# Autodesk Inventor assembly: Heat Exchanger
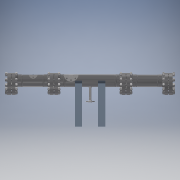
[picture p0: Inventor's stored thumbnail of the model, 180x180]
Saved by Autodesk Inventor 2016 (Build 200138000, 138)
## iProperties
Created: 2018-11-05
Part Number: Heat Exchanger
Document SubType Name: Weldment
Designer: Wijaya
Weld Material: Steel, Carbon
Mass: 1.24439e+06 g
Surface Area: 233524 cm^2
Volume: 160879 cm^3
Density: 7.73496 g/cm^3
_SolveAssemblyDoc: Frame Generator Solve Assembly
_Version: 15.0.0
Author: Wijaya
## Documents named in this file (30)
- C:\Users\Wijaya\Documents\Inventor\Medcom\Heat Exchanger.iam
- C:\Users\Wijaya\Documents\Inventor\Medcom\Shell Pipe.ipt
- C:\Users\Wijaya\Documents\Inventor\Medcom\Weldneck Flange 14 in.ipt
- C:\Users\Wijaya\Documents\Inventor\Medcom\Front Head Pipe.ipt
- C:\Users\Wijaya\Documents\Inventor\Content Center Files\R2016\en-US\ASTM F436(1)\ASTM F436 - 1 1_8(1).ipt
- C:\Users\Wijaya\Documents\Inventor\Medcom\Blind Flange 14 in.ipt
- C:\Users\Wijaya\Documents\Inventor\Medcom\Gasket.ipt
- C:\Users\Wijaya\Documents\Inventor\Medcom\Rear Head Pipe.ipt
- C:\Users\Wijaya\Documents\Inventor\Medcom\Lifting Lug.ipt
- C:\Users\Wijaya\Documents\Inventor\Medcom\Fix Saddle.ipt
- C:\Users\Wijaya\Documents\Inventor\Medcom\Slidding Saddle.ipt
- C:\Users\Wijaya\Documents\Inventor\Medcom\Tube.ipt
- C:\Users\Wijaya\Documents\Inventor\Medcom\Tube Sheet.ipt
- C:\Users\Wijaya\Documents\Inventor\Medcom\Heat Exchanger\Frame\Frame0002.iam
- C:\Users\Wijaya\Documents\Inventor\Medcom\Heat Exchanger\Frame\Frame00021.iam
- C:\Users\Wijaya\Documents\Inventor\Medcom\Tie Rod.ipt
- C:\Users\Wijaya\Documents\Inventor\Medcom\Flange 3 in.ipt
- C:\Users\Wijaya\Documents\Inventor\Medcom\Flange 1 in.ipt
- C:\Users\Wijaya\Documents\Inventor\Medcom\Plate Partition.ipt
- C:\Users\Wijaya\Documents\Inventor\Medcom\Nozzle Pipe 3 in.ipt
- C:\Users\Wijaya\Documents\Inventor\Medcom\Nozzle Pipe 1 in.ipt
- C:\Users\Wijaya\Documents\Inventor\Medcom\Nozzle Pipe 1 in drain.ipt
- C:\Users\Wijaya\Documents\Inventor\Medcom\DIN 976-1 - M30 x 180 - A.ipt
- C:\Users\Wijaya\Documents\Inventor\Medcom\DIN 6915 - M30.ipt
- C:\Users\Wijaya\Documents\Inventor\Medcom\Heat Exchanger\AIP\FEA\cpcsafi80.fins
- C:\Users\Wijaya\Documents\Inventor\Medcom\Heat Exchanger\AIP\FEA\cpcsafi80.fsat
- C:\Users\Wijaya\Documents\Inventor\Medcom\Heat Exchanger\AIP\FEA\cpcsafi80.ftes
- C:\Users\Wijaya\Documents\Inventor\Medcom\Heat Exchanger\AIP\FEA\cpcsafi80.fwiz
- C:\Users\Wijaya\Documents\Inventor\Medcom\Heat Exchanger\AIP\FEA\cpcsafj28.fmsh
- C:\Users\Wijaya\Documents\Inventor\Medcom\Heat Exchanger\AIP\FEA\cpcsafj29.fres
## Components (439 placed, 23 different names)
1. Shell Pipe:1 — Mate:3, Mate:4, Mate:12, Mate:14, Mate:15, Mate:18, Mate:19, Mate:42, Mate:61, Mate:77, Mate:78, Mate:79, Mate:80, Mate:101, Flush:1, Mate:103, Flush:2, Mate:106, Mate:107, Mate:108, Mate:109, Mate:117, Mate:118, Mate:119, Mate:120, Mate:141, Mate:142, Mate:146, Mate:147, Mate:161, Mate:162
2. Weldneck Flange 14 in:1 — Mate:118, Mate:119, Mate:120, Mate:121, Mate:122, Flush:6, Mate:123, Symmetry:5, Rotational:8
3. Weldneck Flange 14 in:2 — Mate:3, Mate:4, Mate:14, Rotational:1, Symmetry:3, Mate:116, Mate:182, Rotational:9
4. Nozzle Pipe 3 in:1 — Mate:141, Mate:142, Mate:143, Mate:144, Mate:145
5. Nozzle Pipe 3 in:2 — Mate:146, Mate:147, Mate:148, Mate:149, Mate:150
6. Nozzle Pipe 1 in drain:1 — Mate:161, Mate:162, Mate:163, Mate:164, Mate:165
7. Flange 3 in:1 — Mate:143, Mate:144, Mate:145
8. Flange 3 in:2 — Mate:148, Mate:149, Mate:150
9. Flange 1 in:3 — Mate:163, Mate:164, Mate:165
10. Plate Partition:1 — Mate:139, Mate:140, Mate:198
11. Gasket:1 — Mate:42, Mate:43, Mate:123
12. Gasket:3 — Rotational:1, Rotational:2
13. Front Head Pipe:1 — Mate:10, Mate:11, Mate:12, Mate:16, Mate:17, Mate:19, Mate:139, Mate:140, Mate:151, Mate:152, Mate:156, Mate:157
14. Weldneck Flange 14 in:3 — Mate:15, Mate:16, Mate:17, Mate:33, Mate:44, Mate:45, Mate:60, Symmetry:2, Mate:170, Mate:173
15. Weldneck Flange 14 in:4 — Mate:10, Mate:11, Mate:18, Mate:43, Mate:174, Symmetry:5, Rotational:7, Mate:180, Mate:181
16. Blind Flange 14 in:1 — Mate:60, Mate:61, Mate:62, Symmetry:2, Mate:65, Mate:166, Mate:198
17. Nozzle Pipe 1 in:1 — Mate:151, Mate:152, Mate:153, Mate:154, Mate:155
18. Nozzle Pipe 1 in:2 — Mate:156, Mate:157, Mate:158, Mate:159, Mate:160
19. Flange 1 in:1 — Mate:153, Mate:154, Mate:155
20. Flange 1 in:2 — Mate:158, Mate:159, Mate:160
21. Gasket:2 — Mate:44, Mate:45, Mate:62
22. Rear Head Pipe:1 — Rotational:3, Rotational:4, Mate:80
23. Weldneck Flange 14 in:5 — Rotational:2, Rotational:3, Mate:77, Symmetry:3, Rotational:10, Mate:186, Mate:189
24. Weldneck Flange 14 in:6 — Rotational:4, Rotational:5, Mate:78, Symmetry:4, Mate:190, Rotational:11, Mate:196, Mate:197
25. Blind Flange 14 in:2 — Rotational:6, Mate:79, Symmetry:4, Rotational:12
26. Gasket:4 — Rotational:5, Rotational:6
27. Lifting Lug:1 — Mate:101, Flush:1, Mate:102
28. Lifting Lug:2 — Mate:103, Flush:2, Mate:104
29. Fix Saddle:1 — Mate:106, Mate:108, Mate:110
30. Slidding Saddle:1 — Mate:107, Mate:109, Mate:111
31. Tube Sheet:1 — Mate:116, Mate:117, Flush:5
32. Tube Sheet:2 — Mate:121, Mate:122, Flush:6, Mate:124, Flush:7
33. Tube:1 — Flush:5
34. Frame0002:1 [sub-assembly]
35. Frame00021:1 [sub-assembly]
36. Tie Rod:1 — Mate:124, Flush:7
37. Tie Rod:2
38. Tie Rod:3
39. Tie Rod:4
40. DIN 976-1 A M30 x 180:1 — Mate:166, Mate:167, Mate:168, Mate:171
41. DIN 6915 M30:1 — Mate:171, Mate:172, Mate:173
42. DIN 6915 M30:2 — Mate:168, Mate:169, Mate:170
43. Circular Washer (Inch) 1 1/8:41 — Mate:33, Mate:169
44. Circular Washer (Inch) 1 1/8:43 — Mate:65, Mate:172
45. DIN 976-1 A M30 x 180:2
46. DIN 6915 M30:3
47. DIN 6915 M30:4
48. Circular Washer (Inch) 1 1/8:44
49. Circular Washer (Inch) 1 1/8:45
50. DIN 976-1 A M30 x 180:3
51. DIN 6915 M30:5
52. DIN 6915 M30:6
53. Circular Washer (Inch) 1 1/8:46
54. Circular Washer (Inch) 1 1/8:47
55. DIN 976-1 A M30 x 180:4
56. DIN 6915 M30:7
57. DIN 6915 M30:8
58. Circular Washer (Inch) 1 1/8:48
59. Circular Washer (Inch) 1 1/8:49
60. DIN 976-1 A M30 x 180:5
61. DIN 6915 M30:9
62. DIN 6915 M30:10
63. Circular Washer (Inch) 1 1/8:50
64. Circular Washer (Inch) 1 1/8:51
65. DIN 976-1 A M30 x 180:6
66. DIN 6915 M30:11
67. DIN 6915 M30:12
68. Circular Washer (Inch) 1 1/8:52
69. Circular Washer (Inch) 1 1/8:53
70. DIN 976-1 A M30 x 180:7
71. DIN 6915 M30:13
72. DIN 6915 M30:14
73. Circular Washer (Inch) 1 1/8:54
74. Circular Washer (Inch) 1 1/8:55
75. DIN 976-1 A M30 x 180:8
76. DIN 6915 M30:15
77. DIN 6915 M30:16
78. Circular Washer (Inch) 1 1/8:56
79. Circular Washer (Inch) 1 1/8:57
80. DIN 976-1 A M30 x 180:9
81. DIN 6915 M30:17
82. DIN 6915 M30:18
83. Circular Washer (Inch) 1 1/8:58
84. Circular Washer (Inch) 1 1/8:59
85. DIN 976-1 A M30 x 180:10
86. DIN 6915 M30:19
87. DIN 6915 M30:20
88. Circular Washer (Inch) 1 1/8:60
89. Circular Washer (Inch) 1 1/8:61
90. DIN 976-1 A M30 x 180:11
91. DIN 6915 M30:21
92. DIN 6915 M30:22
93. Circular Washer (Inch) 1 1/8:62
94. Circular Washer (Inch) 1 1/8:63
95. DIN 976-1 A M30 x 180:12
96. DIN 6915 M30:23
97. DIN 6915 M30:24
98. Circular Washer (Inch) 1 1/8:64
99. Circular Washer (Inch) 1 1/8:65
100. DIN 976-1 A M30 x 180:13
101. DIN 6915 M30:25
102. DIN 6915 M30:26
103. Circular Washer (Inch) 1 1/8:66
104. Circular Washer (Inch) 1 1/8:67
105. DIN 976-1 A M30 x 180:14
106. DIN 6915 M30:27
107. DIN 6915 M30:28
108. Circular Washer (Inch) 1 1/8:68
109. Circular Washer (Inch) 1 1/8:69
110. DIN 976-1 A M30 x 180:15
111. DIN 6915 M30:29
112. DIN 6915 M30:30
113. Circular Washer (Inch) 1 1/8:70
114. Circular Washer (Inch) 1 1/8:71
115. DIN 976-1 A M30 x 180:16
116. DIN 6915 M30:31
117. DIN 6915 M30:32
118. Circular Washer (Inch) 1 1/8:72
119. Circular Washer (Inch) 1 1/8:73
120. DIN 976-1 A M30 x 180:17
121. DIN 6915 M30:33
122. DIN 6915 M30:34
123. Circular Washer (Inch) 1 1/8:74
124. Circular Washer (Inch) 1 1/8:75
125. DIN 976-1 A M30 x 180:18
126. DIN 6915 M30:35
127. DIN 6915 M30:36
128. Circular Washer (Inch) 1 1/8:76
129. Circular Washer (Inch) 1 1/8:77
130. DIN 976-1 A M30 x 180:19
131. DIN 6915 M30:37
132. DIN 6915 M30:38
133. Circular Washer (Inch) 1 1/8:78
134. Circular Washer (Inch) 1 1/8:79
135. DIN 976-1 A M30 x 180:20
136. DIN 6915 M30:39
137. DIN 6915 M30:40
138. Circular Washer (Inch) 1 1/8:80
139. Circular Washer (Inch) 1 1/8:81
140. DIN 976-1 A M30 x 180:21 — Mate:174, Mate:175, Mate:176, Mate:177
141. DIN 6915 M30:41 — Mate:176, Mate:179, Mate:180
142. DIN 6915 M30:42 — Mate:177, Mate:178, Mate:181
143. Circular Washer (Inch) 1 1/8:82 — Rotational:7, Mate:179
144. Circular Washer (Inch) 1 1/8:83 — Rotational:8, Mate:178
145. DIN 976-1 A M30 x 180:24
146. DIN 6915 M30:47
147. DIN 6915 M30:48
148. Circular Washer (Inch) 1 1/8:88
149. Circular Washer (Inch) 1 1/8:89
150. DIN 976-1 A M30 x 180:25
151. DIN 6915 M30:49
152. DIN 6915 M30:50
153. Circular Washer (Inch) 1 1/8:90
154. Circular Washer (Inch) 1 1/8:91
155. DIN 976-1 A M30 x 180:26
156. DIN 6915 M30:51
157. DIN 6915 M30:52
158. Circular Washer (Inch) 1 1/8:92
159. Circular Washer (Inch) 1 1/8:93
160. DIN 976-1 A M30 x 180:27
161. DIN 6915 M30:53
162. DIN 6915 M30:54
163. Circular Washer (Inch) 1 1/8:94
164. Circular Washer (Inch) 1 1/8:95
165. DIN 976-1 A M30 x 180:28
166. DIN 6915 M30:55
167. DIN 6915 M30:56
168. Circular Washer (Inch) 1 1/8:96
169. Circular Washer (Inch) 1 1/8:97
170. DIN 976-1 A M30 x 180:29
171. DIN 6915 M30:57
172. DIN 6915 M30:58
173. Circular Washer (Inch) 1 1/8:98
174. Circular Washer (Inch) 1 1/8:99
175. DIN 976-1 A M30 x 180:30
176. DIN 6915 M30:59
177. DIN 6915 M30:60
178. Circular Washer (Inch) 1 1/8:100
179. Circular Washer (Inch) 1 1/8:101
180. DIN 976-1 A M30 x 180:31
181. DIN 6915 M30:61
182. DIN 6915 M30:62
183. Circular Washer (Inch) 1 1/8:102
184. Circular Washer (Inch) 1 1/8:103
185. DIN 976-1 A M30 x 180:32
186. DIN 6915 M30:63
187. DIN 6915 M30:64
188. Circular Washer (Inch) 1 1/8:104
189. Circular Washer (Inch) 1 1/8:105
190. DIN 976-1 A M30 x 180:33
191. DIN 6915 M30:65
192. DIN 6915 M30:66
193. Circular Washer (Inch) 1 1/8:106
194. Circular Washer (Inch) 1 1/8:107
195. DIN 976-1 A M30 x 180:34
196. DIN 6915 M30:67
197. DIN 6915 M30:68
198. Circular Washer (Inch) 1 1/8:108
199. Circular Washer (Inch) 1 1/8:109
200. DIN 976-1 A M30 x 180:35
201. DIN 6915 M30:69
202. DIN 6915 M30:70
203. Circular Washer (Inch) 1 1/8:110
204. Circular Washer (Inch) 1 1/8:111
205. DIN 976-1 A M30 x 180:36
206. DIN 6915 M30:71
207. DIN 6915 M30:72
208. Circular Washer (Inch) 1 1/8:112
209. Circular Washer (Inch) 1 1/8:113
210. DIN 976-1 A M30 x 180:37
211. DIN 6915 M30:73
212. DIN 6915 M30:74
213. Circular Washer (Inch) 1 1/8:114
214. Circular Washer (Inch) 1 1/8:115
215. DIN 976-1 A M30 x 180:38
216. DIN 6915 M30:75
217. DIN 6915 M30:76
218. Circular Washer (Inch) 1 1/8:116
219. Circular Washer (Inch) 1 1/8:117
220. DIN 976-1 A M30 x 180:39
221. DIN 6915 M30:77
222. DIN 6915 M30:78
223. Circular Washer (Inch) 1 1/8:118
224. Circular Washer (Inch) 1 1/8:119
225. DIN 976-1 A M30 x 180:40
226. DIN 6915 M30:79
227. DIN 6915 M30:80
228. Circular Washer (Inch) 1 1/8:120
229. Circular Washer (Inch) 1 1/8:121
230. DIN 976-1 A M30 x 180:41
231. DIN 6915 M30:81
232. DIN 6915 M30:82
233. Circular Washer (Inch) 1 1/8:122
234. Circular Washer (Inch) 1 1/8:123
235. DIN 976-1 A M30 x 180:42
236. DIN 6915 M30:83
237. DIN 6915 M30:84
238. Circular Washer (Inch) 1 1/8:124
239. Circular Washer (Inch) 1 1/8:125
240. Circular Washer (Inch) 1 1/8:84 — Rotational:9, Mate:185
241. Circular Washer (Inch) 1 1/8:85 — Rotational:10, Mate:188
242. DIN 976-1 A M30 x 180:22 — Mate:182, Mate:183, Mate:184, Mate:187
243. DIN 6915 M30:43 — Mate:184, Mate:185, Mate:186
244. DIN 6915 M30:45 — Mate:187, Mate:188, Mate:189
245. Circular Washer (Inch) 1 1/8:126
246. Circular Washer (Inch) 1 1/8:127
247. DIN 976-1 A M30 x 180:43
248. DIN 6915 M30:85
249. DIN 6915 M30:86
250. Circular Washer (Inch) 1 1/8:128
251. Circular Washer (Inch) 1 1/8:129
252. DIN 976-1 A M30 x 180:44
253. DIN 6915 M30:87
254. DIN 6915 M30:88
255. Circular Washer (Inch) 1 1/8:130
256. Circular Washer (Inch) 1 1/8:131
257. DIN 976-1 A M30 x 180:45
258. DIN 6915 M30:89
259. DIN 6915 M30:90
260. Circular Washer (Inch) 1 1/8:132
261. Circular Washer (Inch) 1 1/8:133
262. DIN 976-1 A M30 x 180:46
263. DIN 6915 M30:91
264. DIN 6915 M30:92
265. Circular Washer (Inch) 1 1/8:134
266. Circular Washer (Inch) 1 1/8:135
267. DIN 976-1 A M30 x 180:47
268. DIN 6915 M30:93
269. DIN 6915 M30:94
270. Circular Washer (Inch) 1 1/8:136
271. Circular Washer (Inch) 1 1/8:137
272. DIN 976-1 A M30 x 180:48
273. DIN 6915 M30:95
274. DIN 6915 M30:96
275. Circular Washer (Inch) 1 1/8:138
276. Circular Washer (Inch) 1 1/8:139
277. DIN 976-1 A M30 x 180:49
278. DIN 6915 M30:97
279. DIN 6915 M30:98
280. Circular Washer (Inch) 1 1/8:140
281. Circular Washer (Inch) 1 1/8:141
282. DIN 976-1 A M30 x 180:50
283. DIN 6915 M30:99
284. DIN 6915 M30:100
285. Circular Washer (Inch) 1 1/8:142
286. Circular Washer (Inch) 1 1/8:143
287. DIN 976-1 A M30 x 180:51
288. DIN 6915 M30:101
289. DIN 6915 M30:102
290. Circular Washer (Inch) 1 1/8:144
291. Circular Washer (Inch) 1 1/8:145
292. DIN 976-1 A M30 x 180:52
293. DIN 6915 M30:103
294. DIN 6915 M30:104
295. Circular Washer (Inch) 1 1/8:146
296. Circular Washer (Inch) 1 1/8:147
297. DIN 976-1 A M30 x 180:53
298. DIN 6915 M30:105
299. DIN 6915 M30:106
300. Circular Washer (Inch) 1 1/8:148
301. Circular Washer (Inch) 1 1/8:149
302. DIN 976-1 A M30 x 180:54
303. DIN 6915 M30:107
304. DIN 6915 M30:108
305. Circular Washer (Inch) 1 1/8:150
306. Circular Washer (Inch) 1 1/8:151
307. DIN 976-1 A M30 x 180:55
308. DIN 6915 M30:109
309. DIN 6915 M30:110
310. Circular Washer (Inch) 1 1/8:152
311. Circular Washer (Inch) 1 1/8:153
312. DIN 976-1 A M30 x 180:56
313. DIN 6915 M30:111
314. DIN 6915 M30:112
315. Circular Washer (Inch) 1 1/8:154
316. Circular Washer (Inch) 1 1/8:155
317. DIN 976-1 A M30 x 180:57
318. DIN 6915 M30:113
319. DIN 6915 M30:114
320. Circular Washer (Inch) 1 1/8:156
321. Circular Washer (Inch) 1 1/8:157
322. DIN 976-1 A M30 x 180:58
323. DIN 6915 M30:115
324. DIN 6915 M30:116
325. Circular Washer (Inch) 1 1/8:158
326. Circular Washer (Inch) 1 1/8:159
327. DIN 976-1 A M30 x 180:59
328. DIN 6915 M30:117
329. DIN 6915 M30:118
330. Circular Washer (Inch) 1 1/8:160
331. Circular Washer (Inch) 1 1/8:161
332. DIN 976-1 A M30 x 180:60
333. DIN 6915 M30:119
334. DIN 6915 M30:120
335. Circular Washer (Inch) 1 1/8:162
336. Circular Washer (Inch) 1 1/8:163
337. DIN 976-1 A M30 x 180:61
338. DIN 6915 M30:121
339. DIN 6915 M30:122
340. Circular Washer (Inch) 1 1/8:86 — Rotational:11, Mate:193
341. Circular Washer (Inch) 1 1/8:87 — Rotational:12, Mate:195
342. DIN 976-1 A M30 x 180:23 — Mate:190, Mate:191, Mate:192, Mate:194
343. DIN 6915 M30:44 — Mate:192, Mate:193, Mate:196
344. DIN 6915 M30:46 — Mate:194, Mate:195, Mate:197
345. Circular Washer (Inch) 1 1/8:164
346. Circular Washer (Inch) 1 1/8:165
347. DIN 976-1 A M30 x 180:62
348. DIN 6915 M30:123
349. DIN 6915 M30:124
350. Circular Washer (Inch) 1 1/8:166
351. Circular Washer (Inch) 1 1/8:167
352. DIN 976-1 A M30 x 180:63
353. DIN 6915 M30:125
354. DIN 6915 M30:126
355. Circular Washer (Inch) 1 1/8:168
356. Circular Washer (Inch) 1 1/8:169
357. DIN 976-1 A M30 x 180:64
358. DIN 6915 M30:127
359. DIN 6915 M30:128
360. Circular Washer (Inch) 1 1/8:170
361. Circular Washer (Inch) 1 1/8:171
362. DIN 976-1 A M30 x 180:65
363. DIN 6915 M30:129
364. DIN 6915 M30:130
365. Circular Washer (Inch) 1 1/8:172
366. Circular Washer (Inch) 1 1/8:173
367. DIN 976-1 A M30 x 180:66
368. DIN 6915 M30:131
369. DIN 6915 M30:132
370. Circular Washer (Inch) 1 1/8:174
371. Circular Washer (Inch) 1 1/8:175
372. DIN 976-1 A M30 x 180:67
373. DIN 6915 M30:133
374. DIN 6915 M30:134
375. Circular Washer (Inch) 1 1/8:176
376. Circular Washer (Inch) 1 1/8:177
377. DIN 976-1 A M30 x 180:68
378. DIN 6915 M30:135
379. DIN 6915 M30:136
380. Circular Washer (Inch) 1 1/8:178
381. Circular Washer (Inch) 1 1/8:179
382. DIN 976-1 A M30 x 180:69
383. DIN 6915 M30:137
384. DIN 6915 M30:138
385. Circular Washer (Inch) 1 1/8:180
386. Circular Washer (Inch) 1 1/8:181
387. DIN 976-1 A M30 x 180:70
388. DIN 6915 M30:139
389. DIN 6915 M30:140
390. Circular Washer (Inch) 1 1/8:182
391. Circular Washer (Inch) 1 1/8:183
392. DIN 976-1 A M30 x 180:71
393. DIN 6915 M30:141
394. DIN 6915 M30:142
395. Circular Washer (Inch) 1 1/8:184
396. Circular Washer (Inch) 1 1/8:185
397. DIN 976-1 A M30 x 180:72
398. DIN 6915 M30:143
399. DIN 6915 M30:144
400. Circular Washer (Inch) 1 1/8:186
401. Circular Washer (Inch) 1 1/8:187
402. DIN 976-1 A M30 x 180:73
403. DIN 6915 M30:145
404. DIN 6915 M30:146
405. Circular Washer (Inch) 1 1/8:188
406. Circular Washer (Inch) 1 1/8:189
407. DIN 976-1 A M30 x 180:74
408. DIN 6915 M30:147
409. DIN 6915 M30:148
410. Circular Washer (Inch) 1 1/8:190
411. Circular Washer (Inch) 1 1/8:191
412. DIN 976-1 A M30 x 180:75
413. DIN 6915 M30:149
414. DIN 6915 M30:150
415. Circular Washer (Inch) 1 1/8:192
416. Circular Washer (Inch) 1 1/8:193
417. DIN 976-1 A M30 x 180:76
418. DIN 6915 M30:151
419. DIN 6915 M30:152
420. Circular Washer (Inch) 1 1/8:194
421. Circular Washer (Inch) 1 1/8:195
422. DIN 976-1 A M30 x 180:77
423. DIN 6915 M30:153
424. DIN 6915 M30:154
425. Circular Washer (Inch) 1 1/8:196
426. Circular Washer (Inch) 1 1/8:197
427. DIN 976-1 A M30 x 180:78
428. DIN 6915 M30:155
429. DIN 6915 M30:156
430. Circular Washer (Inch) 1 1/8:198
431. Circular Washer (Inch) 1 1/8:199
432. DIN 976-1 A M30 x 180:79
433. DIN 6915 M30:157
434. DIN 6915 M30:158
435. Circular Washer (Inch) 1 1/8:200
436. Circular Washer (Inch) 1 1/8:201
437. DIN 976-1 A M30 x 180:80
438. DIN 6915 M30:159
439. DIN 6915 M30:160
## Component patterns: (4 elements, first: Tie Rod:1), (20 elements, first: DIN 976-1 A M30 x 180:1 + DIN 6915 M30:1 + DIN 6915 M30:2 + Circular Washer (Inch) 1 1/8:41 + Circular Washer (Inch) 1 1/8:43), (20 elements, first: DIN 976-1 A M30 x 180:21 + DIN 6915 M30:41 + DIN 6915 M30:42 + Circular Washer (Inch) 1 1/8:82 + Circular Washer (Inch) 1 1/8:83), (20 elements, first: Circular Washer (Inch) 1 1/8:84 + Circular Washer (Inch) 1 1/8:85 + DIN 976-1 A M30 x 180:22 + DIN 6915 M30:43 + DIN 6915 M30:45), (20 elements, first: Circular Washer (Inch) 1 1/8:86 + Circular Washer (Inch) 1 1/8:87 + DIN 976-1 A M30 x 180:23 + DIN 6915 M30:44 + DIN 6915 M30:46)
## Relationships (124: Mate 103, RevoluteJoint 12, Flush 5, Symmetry 4)
- Mate:3 (3 mm): Shell Pipe:1 ↔ Weldneck Flange 14 in:2
- Mate:4: Shell Pipe:1 ↔ Weldneck Flange 14 in:2
- Mate:10 (3 mm): Front Head Pipe:1 ↔ Weldneck Flange 14 in:4
- Mate:11: Front Head Pipe:1 ↔ Weldneck Flange 14 in:4
- Mate:12: Shell Pipe:1 ↔ Front Head Pipe:1
- Mate:14: Shell Pipe:1 ↔ Weldneck Flange 14 in:2
- Mate:15: Shell Pipe:1 ↔ Weldneck Flange 14 in:3
- Mate:16 (3 mm): Front Head Pipe:1 ↔ Weldneck Flange 14 in:3
- Mate:17: Front Head Pipe:1 ↔ Weldneck Flange 14 in:3
- Mate:18: Shell Pipe:1 ↔ Weldneck Flange 14 in:4
- Mate:19: Shell Pipe:1 ↔ Front Head Pipe:1
- Mate:33: Weldneck Flange 14 in:3 ↔ Circular Washer (Inch) 1 1/8:41
- Mate:42: Shell Pipe:1 ↔ Gasket:1
- Mate:43: Gasket:1 ↔ Weldneck Flange 14 in:4
- Mate:44: Weldneck Flange 14 in:3 ↔ Gasket:2
- Mate:45: Weldneck Flange 14 in:3 ↔ Gasket:2
- Mate:60: Weldneck Flange 14 in:3 ↔ Blind Flange 14 in:1
- Mate:61: Shell Pipe:1 ↔ Blind Flange 14 in:1
- Mate:62: Blind Flange 14 in:1 ↔ Gasket:2
- Symmetry:2: Weldneck Flange 14 in:3 ↔ Blind Flange 14 in:1
- Mate:65: Blind Flange 14 in:1 ↔ Circular Washer (Inch) 1 1/8:43
- Rotational:1 [RevoluteJoint]: Weldneck Flange 14 in:2 ↔ Gasket:3
- Rotational:2 [RevoluteJoint]: Gasket:3 ↔ Weldneck Flange 14 in:5
- Rotational:3 [RevoluteJoint] (3 mm): Rear Head Pipe:1 ↔ Weldneck Flange 14 in:5
- Rotational:4 [RevoluteJoint] (3 mm): Rear Head Pipe:1 ↔ Weldneck Flange 14 in:6
- Rotational:5 [RevoluteJoint]: Weldneck Flange 14 in:6 ↔ Gasket:4
- Rotational:6 [RevoluteJoint]: Blind Flange 14 in:2 ↔ Gasket:4
- Mate:77: Shell Pipe:1 ↔ Weldneck Flange 14 in:5
- Mate:78: Shell Pipe:1 ↔ Weldneck Flange 14 in:6
- Mate:79: Shell Pipe:1 ↔ Blind Flange 14 in:2
- Mate:80: Shell Pipe:1 ↔ Rear Head Pipe:1
- Symmetry:3: Weldneck Flange 14 in:2 ↔ Weldneck Flange 14 in:5
- Symmetry:4: Weldneck Flange 14 in:6 ↔ Blind Flange 14 in:2
- Mate:101: Shell Pipe:1 ↔ Lifting Lug:1
- Flush:1: Shell Pipe:1 ↔ Lifting Lug:1
- Mate:102 (-249 mm): Lifting Lug:1
- Mate:103: Shell Pipe:1 ↔ Lifting Lug:2
- Flush:2: Shell Pipe:1 ↔ Lifting Lug:2
- Mate:104 (-763 mm): Lifting Lug:2
- Mate:106: Shell Pipe:1 ↔ Fix Saddle:1
- Mate:107: Shell Pipe:1 ↔ Slidding Saddle:1
- Mate:108: Shell Pipe:1 ↔ Fix Saddle:1
- Mate:109: Shell Pipe:1 ↔ Slidding Saddle:1
- Mate:110 (-344 mm): Fix Saddle:1
- Mate:111 (-668 mm): Slidding Saddle:1
- Mate:116: Weldneck Flange 14 in:2 ↔ Tube Sheet:1
- Mate:117: Shell Pipe:1 ↔ Tube Sheet:1
- Flush:5: Tube Sheet:1 ↔ Tube:1
- Mate:118: Shell Pipe:1 ↔ Weldneck Flange 14 in:1
- Mate:119: Shell Pipe:1 ↔ Weldneck Flange 14 in:1
- Mate:120 (3 mm): Shell Pipe:1 ↔ Weldneck Flange 14 in:1
- Mate:121: Weldneck Flange 14 in:1 ↔ Tube Sheet:2
- Mate:122: Weldneck Flange 14 in:1 ↔ Tube Sheet:2
- Flush:6: Weldneck Flange 14 in:1 ↔ Tube Sheet:2
- Mate:123: Weldneck Flange 14 in:1 ↔ Gasket:1
- Mate:124: Tube Sheet:2 ↔ Tie Rod:1
- Flush:7: Tube Sheet:2 ↔ Tie Rod:1
- Mate:139: Plate Partition:1 ↔ Front Head Pipe:1
- Mate:140: Plate Partition:1 ↔ Front Head Pipe:1
- Mate:141: Shell Pipe:1 ↔ Nozzle Pipe 3 in:1
- Mate:142: Shell Pipe:1 ↔ Nozzle Pipe 3 in:1
- Mate:143 (3 mm): Nozzle Pipe 3 in:1 ↔ Flange 3 in:1
- Mate:144: Nozzle Pipe 3 in:1 ↔ Flange 3 in:1
- Mate:145: Nozzle Pipe 3 in:1 ↔ Flange 3 in:1
- Mate:146: Shell Pipe:1 ↔ Nozzle Pipe 3 in:2
- Mate:147: Shell Pipe:1 ↔ Nozzle Pipe 3 in:2
- Mate:148 (3 mm): Nozzle Pipe 3 in:2 ↔ Flange 3 in:2
- Mate:149: Nozzle Pipe 3 in:2 ↔ Flange 3 in:2
- Mate:150: Nozzle Pipe 3 in:2 ↔ Flange 3 in:2
- Mate:151: Front Head Pipe:1 ↔ Nozzle Pipe 1 in:1
- Mate:152: Front Head Pipe:1 ↔ Nozzle Pipe 1 in:1
- Mate:153 (3 mm): Nozzle Pipe 1 in:1 ↔ Flange 1 in:1
- Mate:154: Nozzle Pipe 1 in:1 ↔ Flange 1 in:1
- Mate:155: Nozzle Pipe 1 in:1 ↔ Flange 1 in:1
- Mate:156: Front Head Pipe:1 ↔ Nozzle Pipe 1 in:2
- Mate:157: Front Head Pipe:1 ↔ Nozzle Pipe 1 in:2
- Mate:158: Nozzle Pipe 1 in:2 ↔ Flange 1 in:2
- Mate:159: Nozzle Pipe 1 in:2 ↔ Flange 1 in:2
- Mate:160 (3 mm): Nozzle Pipe 1 in:2 ↔ Flange 1 in:2
- Mate:161: Shell Pipe:1 ↔ Nozzle Pipe 1 in drain:1
- Mate:162: Shell Pipe:1 ↔ Nozzle Pipe 1 in drain:1
- Mate:163: Nozzle Pipe 1 in drain:1 ↔ Flange 1 in:3
- Mate:164 (3 mm): Nozzle Pipe 1 in drain:1 ↔ Flange 1 in:3
- Mate:165: Nozzle Pipe 1 in drain:1 ↔ Flange 1 in:3
- Mate:166: Blind Flange 14 in:1 ↔ DIN 976-1 A M30 x 180:1
- Mate:167: DIN 976-1 A M30 x 180:1
- Mate:168: DIN 976-1 A M30 x 180:1 ↔ DIN 6915 M30:2
- Mate:169: DIN 6915 M30:2 ↔ Circular Washer (Inch) 1 1/8:41
- Mate:170: Weldneck Flange 14 in:3 ↔ DIN 6915 M30:2
- Mate:171: DIN 976-1 A M30 x 180:1 ↔ DIN 6915 M30:1
- Mate:172: DIN 6915 M30:1 ↔ Circular Washer (Inch) 1 1/8:43
- Mate:173: Weldneck Flange 14 in:3 ↔ DIN 6915 M30:1
- Mate:174: Weldneck Flange 14 in:4 ↔ DIN 976-1 A M30 x 180:21
- Symmetry:5: Weldneck Flange 14 in:1 ↔ Weldneck Flange 14 in:4
- Mate:175: DIN 976-1 A M30 x 180:21
- Rotational:7 [RevoluteJoint]: Weldneck Flange 14 in:4 ↔ Circular Washer (Inch) 1 1/8:82
- Rotational:8 [RevoluteJoint]: Weldneck Flange 14 in:1 ↔ Circular Washer (Inch) 1 1/8:83
- Mate:176: DIN 976-1 A M30 x 180:21 ↔ DIN 6915 M30:41
- Mate:177: DIN 976-1 A M30 x 180:21 ↔ DIN 6915 M30:42
- Mate:178: DIN 6915 M30:42 ↔ Circular Washer (Inch) 1 1/8:83
- Mate:179: DIN 6915 M30:41 ↔ Circular Washer (Inch) 1 1/8:82
- Mate:180: Weldneck Flange 14 in:4 ↔ DIN 6915 M30:41
- Mate:181: Weldneck Flange 14 in:4 ↔ DIN 6915 M30:42
- Mate:182: Weldneck Flange 14 in:2 ↔ DIN 976-1 A M30 x 180:22
- Mate:183: DIN 976-1 A M30 x 180:22
- Rotational:9 [RevoluteJoint]: Weldneck Flange 14 in:2 ↔ Circular Washer (Inch) 1 1/8:84
- Rotational:10 [RevoluteJoint]: Weldneck Flange 14 in:5 ↔ Circular Washer (Inch) 1 1/8:85
- Mate:184: DIN 976-1 A M30 x 180:22 ↔ DIN 6915 M30:43
- Mate:185: Circular Washer (Inch) 1 1/8:84 ↔ DIN 6915 M30:43
- Mate:186: Weldneck Flange 14 in:5 ↔ DIN 6915 M30:43
- Mate:187: DIN 976-1 A M30 x 180:22 ↔ DIN 6915 M30:45
- Mate:188: Circular Washer (Inch) 1 1/8:85 ↔ DIN 6915 M30:45
- Mate:189: Weldneck Flange 14 in:5 ↔ DIN 6915 M30:45
- Mate:190: Weldneck Flange 14 in:6 ↔ DIN 976-1 A M30 x 180:23
- Mate:191: DIN 976-1 A M30 x 180:23
- Rotational:11 [RevoluteJoint]: Weldneck Flange 14 in:6 ↔ Circular Washer (Inch) 1 1/8:86
- Rotational:12 [RevoluteJoint]: Blind Flange 14 in:2 ↔ Circular Washer (Inch) 1 1/8:87
- Mate:192: DIN 976-1 A M30 x 180:23 ↔ DIN 6915 M30:44
- Mate:193: Circular Washer (Inch) 1 1/8:86 ↔ DIN 6915 M30:44
- Mate:194: DIN 976-1 A M30 x 180:23 ↔ DIN 6915 M30:46
- Mate:195: Circular Washer (Inch) 1 1/8:87 ↔ DIN 6915 M30:46
- Mate:196: Weldneck Flange 14 in:6 ↔ DIN 6915 M30:44
- Mate:197: Weldneck Flange 14 in:6 ↔ DIN 6915 M30:46
- Mate:198: Plate Partition:1 ↔ Blind Flange 14 in:1
## Named parameters: sa_0 = 0, sa_1 = 0, sa_2 = -980.6, sa_3 = 20680, sa_4 = 20680
note: some values were not read from the file. Shown as the stored number, unit unknown: "sa_0", "sa_1", "sa_2", "sa_3", "sa_4".
